# Autodesk Inventor assembly: 20-J2
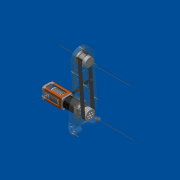
[picture p0: Inventor's stored thumbnail of the model, 180x180]
Saved by Autodesk Inventor 2018 (Build 220112000, 112)
## iProperties
Created: 2020-01-14
Part Number: 20-J2
Document SubType Name: Assembly
Designer: Bunny320
Author: Bunny320
## Documents named in this file (12)
- C:\Users\Bunny320\Desktop\sechs\4-CAD\30-J3.iam
- C:\Users\Bunny320\Desktop\sechs\4-CAD\201-flange-with motor.ipt
- C:\Users\Bunny320\Desktop\sechs\4-CAD\standardParts\61807-2RS1\61807-2RS1.iam
- C:\Users\Bunny320\Desktop\sechs\4-CAD\motor unit.iam
- C:\Users\Bunny320\Desktop\sechs\4-CAD\303-link right.ipt
- C:\Users\Bunny320\Desktop\sechs\4-CAD\generated\J3_belt.iam
- C:\Users\Bunny320\Documents\Inventor\Content Center Files\R2018\en-US\ISO 10642(2)\ISO 10642  - M4  x  20.ipt
- C:\Users\Bunny320\Documents\Inventor\Content Center Files\R2018\en-US\ISO 4762(1)\DIN EN ISO 4762 - M3 x 12.ipt
- C:\Users\Bunny320\Documents\Inventor\Content Center Files\R2018\en-US\ISO 4762(1)\DIN EN ISO 4762 - M3 x 20.ipt
- C:\Users\Bunny320\Documents\Inventor\Content Center Files\R2018\en-US\DIN EN ISO 4032\DIN EN ISO 4032 - M3.ipt
- C:\Users\Bunny320\Documents\Inventor\Content Center Files\R2018\en-US\ISO 4762(1)\DIN EN ISO 4762 - M3 x 25.ipt
- C:\Users\Bunny320\Desktop\sechs\4-CAD\standardParts\Pololu mounting hub\pololu-universal-aluminum-mounting-hub-for-8mm-shaft-m3-holes.ipt
## Components (23 placed, 11 different names)
1. 201-flange-with motor:1 — Flush:1, Flush:2, Flush:3, Mate:3, Mate:4, Mate:7, Mate:8, Mate:9, Mate:22, Mate:23, Mate:24, Mate:25, Mate:34, Mate:35, Mate:36, Mate:37, Mate:38, Mate:39, Mate:40, Mate:41, Mate:42, Mate:43, Insert:1
2. 61807-2RS1:1 [sub-assembly] — Mate:3, Mate:4, Mate:10, Mate:58
3. 61807-2RS1:2 [sub-assembly] — Mate:12, Mate:13
4. motor unit:1 [sub-assembly] — Mate:7, Mate:8, Mate:9, Mate:14, Mate:56
5. 303-link right:1 — Mate:10, Mate:12, Mate:13, Flush:4, Mate:17, Mate:44, Mate:45, Mate:46, Mate:47, Mate:48, Mate:49, Mate:50, Mate:51, Mate:52, Mate:53, Mate:54, Mate:55, Mate:58
6. J3_belt:1 [sub-assembly] — Flush:4, Mate:14, Mate:17, Mate:57
7. DIN EN ISO 10642 M4  x  20:1 — Mate:22
8. DIN EN ISO 10642 M4  x  20:2 — Mate:23
9. DIN EN ISO 10642 M4  x  20:3 — Mate:24
10. DIN EN ISO 10642 M4  x  20:4 — Mate:25
11. DIN EN ISO 4762 M3 x 12:5 — Mate:34, Mate:35
12. DIN EN ISO 4762 M3 x 12:6 — Mate:36, Mate:37
13. DIN EN ISO 4762 M3 x 12:7 — Mate:38, Mate:39
14. DIN EN ISO 4762 M3 x 12:8 — Mate:40, Mate:41
15. DIN EN ISO 4762 M3 x 20:1 — Mate:42, Mate:43
16. DIN EN ISO 4032 M3:1 — Insert:1
17. DIN EN ISO 4762 M3 x 25:1 — Mate:44, Mate:45
18. DIN EN ISO 4762 M3 x 25:2 — Mate:46, Mate:47
19. DIN EN ISO 4762 M3 x 25:3 — Mate:48, Mate:49
20. DIN EN ISO 4762 M3 x 25:4 — Mate:50, Mate:51
21. DIN EN ISO 4762 M3 x 25:5 — Mate:52, Mate:53
22. DIN EN ISO 4762 M3 x 25:6 — Mate:54, Mate:55
23. pololu-universal-aluminum-mounting-hub-for-8mm-shaft-m3-holes:1 — Mate:56, Mate:57
## Relationships (44: Mate 39, Flush 4, Insert 1)
- Flush:1: 201-flange-with motor:1
- Flush:2: 201-flange-with motor:1
- Flush:3: 201-flange-with motor:1
- Mate:3: 201-flange-with motor:1 ↔ 61807-2RS1:1
- Mate:4: 201-flange-with motor:1 ↔ 61807-2RS1:1
- Mate:7: 201-flange-with motor:1 ↔ motor unit:1
- Mate:8: 201-flange-with motor:1 ↔ motor unit:1
- Mate:9: 201-flange-with motor:1 ↔ motor unit:1
- Mate:10: 61807-2RS1:1 ↔ 303-link right:1
- Mate:12: 61807-2RS1:2 ↔ 303-link right:1
- Mate:13: 61807-2RS1:2 ↔ 303-link right:1
- Flush:4: 303-link right:1 ↔ J3_belt:1
- Mate:14: motor unit:1 ↔ J3_belt:1
- Mate:17: 303-link right:1 ↔ J3_belt:1
- Mate:22: 201-flange-with motor:1 ↔ DIN EN ISO 10642 M4  x  20:1
- Mate:23: 201-flange-with motor:1 ↔ DIN EN ISO 10642 M4  x  20:2
- Mate:24: 201-flange-with motor:1 ↔ DIN EN ISO 10642 M4  x  20:3
- Mate:25: 201-flange-with motor:1 ↔ DIN EN ISO 10642 M4  x  20:4
- Mate:34: 201-flange-with motor:1 ↔ DIN EN ISO 4762 M3 x 12:5
- Mate:35: 201-flange-with motor:1 ↔ DIN EN ISO 4762 M3 x 12:5
- Mate:36: 201-flange-with motor:1 ↔ DIN EN ISO 4762 M3 x 12:6
- Mate:37: 201-flange-with motor:1 ↔ DIN EN ISO 4762 M3 x 12:6
- Mate:38: 201-flange-with motor:1 ↔ DIN EN ISO 4762 M3 x 12:7
- Mate:39: 201-flange-with motor:1 ↔ DIN EN ISO 4762 M3 x 12:7
- Mate:40: 201-flange-with motor:1 ↔ DIN EN ISO 4762 M3 x 12:8
- Mate:41: 201-flange-with motor:1 ↔ DIN EN ISO 4762 M3 x 12:8
- Mate:42: 201-flange-with motor:1 ↔ DIN EN ISO 4762 M3 x 20:1
- Mate:43: 201-flange-with motor:1 ↔ DIN EN ISO 4762 M3 x 20:1
- Insert:1: 201-flange-with motor:1 ↔ DIN EN ISO 4032 M3:1
- Mate:44: 303-link right:1 ↔ DIN EN ISO 4762 M3 x 25:1
- Mate:45: 303-link right:1 ↔ DIN EN ISO 4762 M3 x 25:1
- Mate:46: 303-link right:1 ↔ DIN EN ISO 4762 M3 x 25:2
- Mate:47: 303-link right:1 ↔ DIN EN ISO 4762 M3 x 25:2
- Mate:48: 303-link right:1 ↔ DIN EN ISO 4762 M3 x 25:3
- Mate:49: 303-link right:1 ↔ DIN EN ISO 4762 M3 x 25:3
- Mate:50: 303-link right:1 ↔ DIN EN ISO 4762 M3 x 25:4
- Mate:51: 303-link right:1 ↔ DIN EN ISO 4762 M3 x 25:4
- Mate:52: 303-link right:1 ↔ DIN EN ISO 4762 M3 x 25:5
- Mate:53: 303-link right:1 ↔ DIN EN ISO 4762 M3 x 25:5
- Mate:54: 303-link right:1 ↔ DIN EN ISO 4762 M3 x 25:6
- Mate:55: 303-link right:1 ↔ DIN EN ISO 4762 M3 x 25:6
- Mate:56: motor unit:1 ↔ pololu-universal-aluminum-mounting-hub-for-8mm-shaft-m3-holes:1
- Mate:57: J3_belt:1 ↔ pololu-universal-aluminum-mounting-hub-for-8mm-shaft-m3-holes:1
- Mate:58: 61807-2RS1:1 ↔ 303-link right:1
